# Autodesk Inventor assembly: Samenstelling_v2
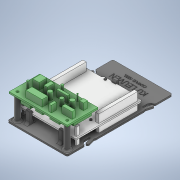
[picture p0: Inventor's stored thumbnail of the model, 180x180]
Saved by Autodesk Inventor 2022 (Build 260153000, 153)
## iProperties
Created: 2022-02-18
Part Number: Samenstelling_v2
Document SubType Name: Assembly
Designer: woutr
Author: woutr
## Documents named in this file (4)
- C:\Users\woutr\OneDrive\Documenten\Inventor\Project Klascomfortmonitoring\Samenstelling_v2.1.iam
- C:\Users\woutr\OneDrive\Documenten\Inventor\Project Klascomfortmonitoring\Microcontroller.ipt
- C:\Users\woutr\OneDrive\Documenten\Inventor\Project Klascomfortmonitoring\printplaat.ipt
- C:\Users\woutr\OneDrive\Documenten\Inventor\Project Klascomfortmonitoring\Bodemplaat_v2.1.ipt
## Components (3 placed, 3 different names)
1. Bodemplaat_v2.1:1 — Mate:1, Mate:2, Mate:3, Mate:4, Mate:5, Mate:6
2. Microcontroller:1 — Mate:1, Mate:2, Mate:3
3. printplaat:1 — Mate:4, Mate:5, Mate:6
## Relationships (6: Mate 6)
- Mate:1: Bodemplaat_v2.1:1 ↔ Microcontroller:1
- Mate:2: Bodemplaat_v2.1:1 ↔ Microcontroller:1
- Mate:3: Bodemplaat_v2.1:1 ↔ Microcontroller:1
- Mate:4: Bodemplaat_v2.1:1 ↔ printplaat:1
- Mate:5: Bodemplaat_v2.1:1 ↔ printplaat:1
- Mate:6: Bodemplaat_v2.1:1 ↔ printplaat:1
